# Autodesk Inventor assembly: Wind Tunnel Settling Chamber
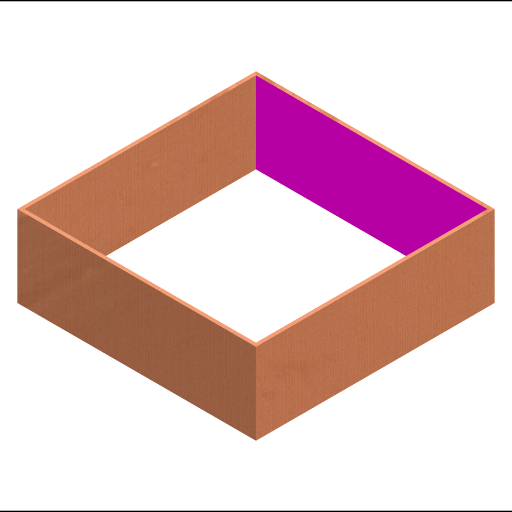
[picture p0: Inventor's stored thumbnail of the model, 512x512]
Saved by Autodesk Inventor 2023 (Build 270158000, 158)
## iProperties
Created: 2022-01-23
Part Number: Wind Tunnel Settling Chamber
Document SubType Name: Assembly
Designer: kamer
Author: kamer
## Documents named in this file (3)
- X:\Storage\Documents\ME 306 Heat Transfer Project Files\CAD\Wind Tunnel Settling Chamber.iam
- X:\Storage\Documents\ME 306 Heat Transfer Project Files\CAD\Wind Tunnel Settling Chamber Side.ipt
- X:\Storage\Documents\ME 306 Heat Transfer Project Files\CAD\Wind Tunnel Settling Chamber Top+Bottom.ipt
## Components (4 placed, 2 different names)
1. Wind Tunnel Settling Chamber Side:1 — Mate:1, Flush:1, Flush:2, Mate:2, Flush:3, Flush:4
2. Wind Tunnel Settling Chamber Top+Bottom:1 — Mate:1, Flush:1, Flush:2
3. Wind Tunnel Settling Chamber Side:2 — Flush:5, Mate:3, Flush:6, Flush:7
4. Wind Tunnel Settling Chamber Top+Bottom:2 — Mate:2, Flush:3, Flush:4, Flush:5, Mate:3, Flush:6, Flush:7
## Relationships (10: Flush 7, Mate 3)
- Mate:1: Wind Tunnel Settling Chamber Side:1 ↔ Wind Tunnel Settling Chamber Top+Bottom:1
- Flush:1: Wind Tunnel Settling Chamber Side:1 ↔ Wind Tunnel Settling Chamber Top+Bottom:1
- Flush:2: Wind Tunnel Settling Chamber Side:1 ↔ Wind Tunnel Settling Chamber Top+Bottom:1
- Mate:2: Wind Tunnel Settling Chamber Side:1 ↔ Wind Tunnel Settling Chamber Top+Bottom:2
- Flush:3: Wind Tunnel Settling Chamber Side:1 ↔ Wind Tunnel Settling Chamber Top+Bottom:2
- Flush:4: Wind Tunnel Settling Chamber Side:1 ↔ Wind Tunnel Settling Chamber Top+Bottom:2
- Flush:5: Wind Tunnel Settling Chamber Side:2 ↔ Wind Tunnel Settling Chamber Top+Bottom:2
- Mate:3: Wind Tunnel Settling Chamber Side:2 ↔ Wind Tunnel Settling Chamber Top+Bottom:2
- Flush:6: Wind Tunnel Settling Chamber Side:2 ↔ Wind Tunnel Settling Chamber Top+Bottom:2
- Flush:7: Wind Tunnel Settling Chamber Side:2 ↔ Wind Tunnel Settling Chamber Top+Bottom:2
